# Autodesk Inventor assembly: Claw Assembly
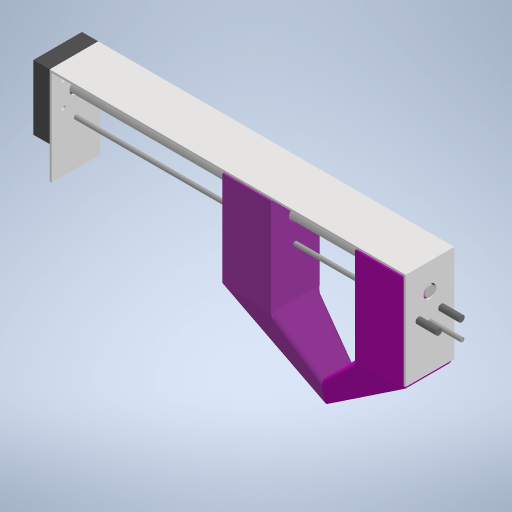
[picture p0: Inventor's stored thumbnail of the model, 512x512]
Saved by Autodesk Inventor 2024 (Build 280153000, 153)
## iProperties
Created: 2025-01-21
Part Number: Claw Assembly
Document SubType Name: Assembly
Designer: Sven
Author: Sven
## Documents named in this file (8)
- C:\Users\Sven\Documents\Inventor\BRC Robotic CLaw\Claw Assembly.iam
- C:\Users\Sven\Documents\Inventor\BRC Robotic CLaw\Bracket.ipt
- C:\Users\Sven\Documents\Inventor\BRC Robotic CLaw\Moving Gripper.ipt
- C:\Users\Sven\Documents\Inventor\BRC Robotic CLaw\Stationary Gripper.ipt
- C:\Users\Sven\Documents\Inventor\BRC Robotic CLaw\Lead Screw.ipt
- C:\Users\Sven\Documents\Inventor\BRC Robotic CLaw\#10 2in.ipt
- C:\Users\Sven\Documents\Inventor\BRC Robotic CLaw\Support Bar.ipt
- C:\Users\Sven\Documents\Inventor\BRC Robotic CLaw\Motor Brace.ipt
## Components (8 placed, 7 different names)
1. Bracket:1 — Mate:3, Flush:1, Mate:4, Mate:5, Mate:12, Mate:13, Mate:15, Flush:2, Mate:17, Mate:18
2. Moving Gripper:1 — Mate:5, Mate:6, Mate:13, Mate:14
3. Stationary Gripper:1 — Mate:4, Mate:7, Mate:8, Mate:9, Mate:10, Mate:11, Mate:12, Mate:14
4. Lead Screw:1 — Mate:3, Flush:1, Mate:6, Mate:7, Mate:16
5. #10 2in:1 — Mate:8, Mate:9
6. #10 2in:2 — Mate:10, Mate:11
7. Support Bar:1 — Mate:15, Flush:2
8. Motor Brace:1 — Mate:16, Mate:17, Mate:18
## Relationships (18: Mate 16, Flush 2)
- Mate:3: Bracket:1 ↔ Lead Screw:1
- Flush:1: Bracket:1 ↔ Lead Screw:1
- Mate:4: Bracket:1 ↔ Stationary Gripper:1
- Mate:5: Bracket:1 ↔ Moving Gripper:1
- Mate:6: Moving Gripper:1 ↔ Lead Screw:1
- Mate:7: Stationary Gripper:1 ↔ Lead Screw:1
- Mate:8: Stationary Gripper:1 ↔ #10 2in:1
- Mate:9: Stationary Gripper:1 ↔ #10 2in:1
- Mate:10: Stationary Gripper:1 ↔ #10 2in:2
- Mate:11: Stationary Gripper:1 ↔ #10 2in:2
- Mate:12: Bracket:1 ↔ Stationary Gripper:1
- Mate:13: Bracket:1 ↔ Moving Gripper:1
- Mate:14: Moving Gripper:1 ↔ Stationary Gripper:1
- Mate:15: Bracket:1 ↔ Support Bar:1
- Flush:2: Bracket:1 ↔ Support Bar:1
- Mate:16: Lead Screw:1 ↔ Motor Brace:1
- Mate:17: Bracket:1 ↔ Motor Brace:1
- Mate:18: Bracket:1 ↔ Motor Brace:1
